# Autodesk Inventor assembly: 06-01-2023 assieme piccolo
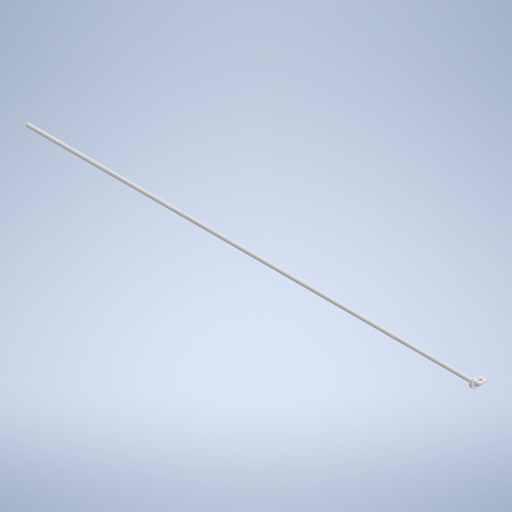
[picture p0: Inventor's stored thumbnail of the model, 512x512]
Saved by Autodesk Inventor 2023 (Build 270158000, 158)
## iProperties
Created: 2023-05-31
Part Number: 06-01-2023 assieme piccolo
Document SubType Name: Assembly
Designer: Admin
Author: Admin
## Documents named in this file (4)
- C:\Users\Admin\Desktop\3DDDD\06-01-2023 assieme piccolo.iam
- C:\Users\Admin\Desktop\3DDDD\06-01-2023 flangia piccola.ipt
- C:\Users\Admin\Desktop\3DDDD\06-01-2023 Verga.ipt
- C:\Users\Admin\Desktop\3DDDD\06-01-2023 curva 90°.ipt
## Components (5 placed, 3 different names)
1. 06-01-2023 flangia piccola:2 — Coincidente:1, Coincidente:2, Coincidente:7, Coincidente:8, Coincidente:9, Coincidente:11, Coincidente:12
2. 06-01-2023 Verga:1 — Coincidente:1, Coincidente:2, Coincidente:10, Coincidente:11
3. 06-01-2023 flangia piccola:3 — Coincidente:3, Coincidente:4, Coincidente:12
4. 06-01-2023 flangia piccola:4 — Coincidente:5, Coincidente:6, Coincidente:7, Coincidente:8, Coincidente:9
5. 06-01-2023 curva 90°:1 — Coincidente:3, Coincidente:4, Coincidente:5, Coincidente:6, Coincidente:10
## Relationships (12: Mate 12)
- Coincidente:1 [Mate]: 06-01-2023 flangia piccola:2 ↔ 06-01-2023 Verga:1
- Coincidente:2 [Mate]: 06-01-2023 flangia piccola:2 ↔ 06-01-2023 Verga:1
- Coincidente:3 [Mate]: 06-01-2023 flangia piccola:3 ↔ 06-01-2023 curva 90°:1
- Coincidente:4 [Mate]: 06-01-2023 flangia piccola:3 ↔ 06-01-2023 curva 90°:1
- Coincidente:5 [Mate]: 06-01-2023 flangia piccola:4 ↔ 06-01-2023 curva 90°:1
- Coincidente:6 [Mate]: 06-01-2023 flangia piccola:4 ↔ 06-01-2023 curva 90°:1
- Coincidente:7 [Mate]: 06-01-2023 flangia piccola:2 ↔ 06-01-2023 flangia piccola:4
- Coincidente:8 [Mate]: 06-01-2023 flangia piccola:2 ↔ 06-01-2023 flangia piccola:4
- Coincidente:9 [Mate]: 06-01-2023 flangia piccola:2 ↔ 06-01-2023 flangia piccola:4
- Coincidente:10 [Mate]: 06-01-2023 Verga:1 ↔ 06-01-2023 curva 90°:1
- Coincidente:11 [Mate]: 06-01-2023 flangia piccola:2 ↔ 06-01-2023 Verga:1
- Coincidente:12 [Mate]: 06-01-2023 flangia piccola:2 ↔ 06-01-2023 flangia piccola:3
